# Autodesk Inventor assembly: Chassie2
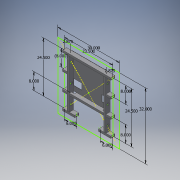
[picture p0: Inventor's stored thumbnail of the model, 180x180]
Saved by Autodesk Inventor 2016 (Build 200138000, 138)
## iProperties
Created: 2017-01-08
Part Number: Chassie2
Document SubType Name: Assembly
Designer: idevr_000
_SolveAssemblyDoc: Frame Generator Solve Assembly
_Version: 15.0.0
Author: idevr_000
## Documents named in this file (4)
- C:\Users\Dhruv\Desktop\MISC\FRC 2017\Chassie2.iam
- C:\Users\Dhruv\Desktop\MISC\FRC 2017\Part602.ipt
- C:\Users\Dhruv\Desktop\MISC\FRC 2017\Chassie2\Frame\Frame0001.iam
- C:\Users\Dhruv\Desktop\MISC\FRC 2017\bellypan.ipt
## Components (3 placed, 3 different names)
1. Part602:1
2. Frame0001:1 [sub-assembly] — Mate:1, Flush:1, Flush:2
3. bellypan:1 — Mate:1, Flush:1, Flush:2
## Relationships (3: Flush 2, Mate 1)
- Mate:1: Frame0001:1 ↔ bellypan:1
- Flush:1: Frame0001:1 ↔ bellypan:1
- Flush:2: Frame0001:1 ↔ bellypan:1
